# Autodesk Inventor assembly: 25mm Stroke Pneumatic Cylinder
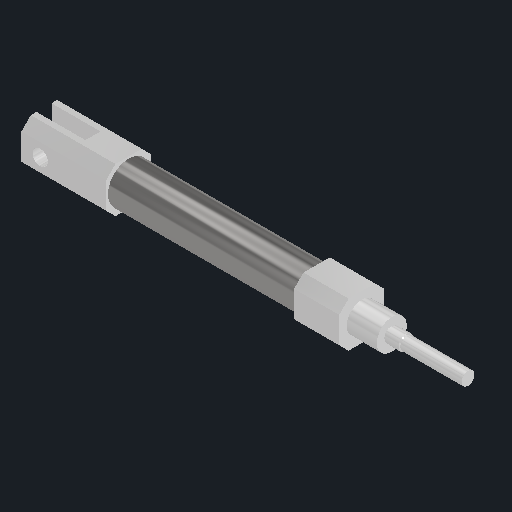
[picture p0: Inventor's stored thumbnail of the model, 512x512]
Saved by Autodesk Inventor 2026.1 (Build 301233000, 233)
## iProperties
Created: 2024-02-02
Part Number: 25mm Stroke Pneumatic Cylinder
Document SubType Name: Assembly
Designer: AdminForWorker
Mass: 9.86623 g
Surface Area: 52.7566 cm^2
Volume: 9.86623 cm^3
Title: 25mm Stroke Pneumatic Cylinder.f3d v1
Author: AdminForWorker
## Documents named in this file (3)
- C:\Users\roejo\OneDrive\Documents\2026WorldChampionRobot\Library\VEX-CAD-Inventor-1.4.2\Motion\Pneumatics\New - V5 Pneumatics\25mm Stroke Pneumatic Cylinder.iam
- C:\Users\roejo\OneDrive\Documents\2026WorldChampionRobot\Library\VEX-CAD-Inventor-1.4.2\Motion\Pneumatics\Reference Parts\Pistons\25mm Stroke Pneumatic Cylinder Body.ipt
- C:\Users\roejo\OneDrive\Documents\2026WorldChampionRobot\Library\VEX-CAD-Inventor-1.4.2\Motion\Pneumatics\Reference Parts\Pistons\25mm Stroke Pneumatic Cylinder Rod.ipt
## Components (2 placed, 2 different names)
1. Component1:1 — Cylindrical:1
2. Component2:1 — Cylindrical:1
## Relationships (1: CylindricalJoint 1)
- Cylindrical:1: Component1:1 ↔ Component2:1
